# Autodesk Inventor assembly: Assembly1
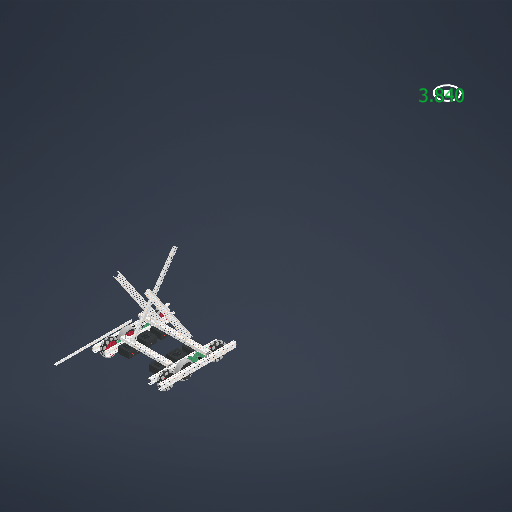
[picture p0: Inventor's stored thumbnail of the model, 512x512]
Saved by Autodesk Inventor 2026.2 (Build 302298000, 298)
## iProperties
Created: 2025-12-27
Part Number: Assembly1
Document SubType Name: Assembly
Designer: jacob
Author: jacob
## Documents named in this file (35)
- C:\Personal\Deprecated\VEX V5 Push Back\S-bot-two\CAD\Assembly1.iam
- C:\Personal\Deprecated\VEX V5 Push Back\S-bot-two\CAD\VEX-CAD-Inventor-1.4.2\Structure\C Channel\Aluminum 1x2x1\Alu C 1x2x1x30.ipt
- C:\Personal\Deprecated\VEX V5 Push Back\S-bot-two\CAD\VEX-CAD-Inventor-1.4.2\Structure\Hardware\Nut Nylock.ipt
- C:\Personal\Deprecated\VEX V5 Push Back\S-bot-two\CAD\VEX-CAD-Inventor-1.4.2\Motion\Spacers\Spacer Nylon .375 OD\NSpacer .375 OD x .500.ipt
- C:\Personal\Deprecated\VEX V5 Push Back\S-bot-two\CAD\VEX-CAD-Inventor-1.4.2\Motion\Spacers\Spacer Nylon .375 OD.ipt
- C:\Personal\Deprecated\VEX V5 Push Back\S-bot-two\CAD\VEX-CAD-Inventor-1.4.2\Motion\Wheels\Omni Wheel\3.25 Omni AS, No Insert.iam
- C:\Personal\Deprecated\VEX V5 Push Back\S-bot-two\CAD\VEX-CAD-Inventor-1.4.2\Motion\Wheels\Omni Wheel.iam
- C:\Personal\Deprecated\VEX V5 Push Back\S-bot-two\CAD\VEX-CAD-Inventor-1.4.2\Motion\HS Shaft Adapter Circle.ipt
- C:\Personal\Deprecated\VEX V5 Push Back\S-bot-two\CAD\VEX-CAD-Inventor-1.4.2\Motion\Wheels\Traction Wheel.iam
- C:\Personal\Deprecated\VEX V5 Push Back\S-bot-two\CAD\VEX-CAD-Inventor-1.4.2\Motion\Spacers\Spacer Nylon .375 OD\NSpacer .375 OD x .125.ipt
- C:\Personal\Deprecated\VEX V5 Push Back\S-bot-two\CAD\VEX-CAD-Inventor-1.4.2\Motion\Spacers\Washer Steel\SWasher .375 OD x .031250.ipt
- C:\Personal\Deprecated\VEX V5 Push Back\S-bot-two\CAD\VEX-CAD-Inventor-1.4.2\Motion\Spacers\Washer Steel.ipt
- C:\Personal\Deprecated\VEX V5 Push Back\S-bot-two\CAD\VEX-CAD-Inventor-1.4.2\Motion\Gears\HS Gear.iam
- C:\Personal\Deprecated\VEX V5 Push Back\S-bot-two\CAD\VEX-CAD-Inventor-1.4.2\Motion\Gears\HS Gear\HS 48T Gear, Circle.iam
- C:\Personal\Deprecated\VEX V5 Push Back\S-bot-two\CAD\VEX-CAD-Inventor-1.4.2\Motion\Gears\LS 36T Gear.ipt
- C:\Personal\Deprecated\VEX V5 Push Back\S-bot-two\CAD\VEX-CAD-Inventor-1.4.2\Structure\C Channel\Aluminum 1x2x1\Alu C 1x2x1x27.ipt
- C:\Personal\Deprecated\VEX V5 Push Back\S-bot-two\CAD\VEX-CAD-Inventor-1.4.2\Electronics\V5 Motor.ipt
- C:\Personal\Deprecated\VEX V5 Push Back\S-bot-two\CAD\VEX-CAD-Inventor-1.4.2\Motion\Shaft LS\Bearing Flat.ipt
- C:\Personal\Deprecated\VEX V5 Push Back\S-bot-two\CAD\VEX-CAD-Inventor-1.4.2\Motion\Spacers\Spacer Nylon .375 OD\NSpacer .375 OD x .250.ipt
- C:\Personal\Deprecated\VEX V5 Push Back\S-bot-two\CAD\VEX-CAD-Inventor-1.4.2\Motion\Wheels\Traction Wheel\3.25 Traction AS, Circle.iam
- C:\Personal\Deprecated\VEX V5 Push Back\S-bot-two\CAD\VEX-CAD-Inventor-1.4.2\Structure\Standoff.ipt
- C:\Personal\Deprecated\VEX V5 Push Back\S-bot-two\CAD\VEX-CAD-Inventor-1.4.2\Structure\Hardware\Nut Nylock_MIR.ipt
- C:\Personal\Deprecated\VEX V5 Push Back\S-bot-two\CAD\VEX-CAD-Inventor-1.4.2\Motion\HS Shaft Adapter Circle_MIR.ipt
- C:\Personal\Deprecated\VEX V5 Push Back\S-bot-two\CAD\VEX-CAD-Inventor-1.4.2\Motion\Gears\LS 36T Gear_MIR.ipt
- C:\Personal\Deprecated\VEX V5 Push Back\S-bot-two\CAD\VEX-CAD-Inventor-1.4.2\Electronics\V5 Motor_MIR.ipt
- C:\Personal\Deprecated\VEX V5 Push Back\S-bot-two\CAD\VEX-CAD-Inventor-1.4.2\Motion\Shaft LS\Bearing Flat_MIR.ipt
- C:\Personal\Deprecated\VEX V5 Push Back\S-bot-two\CAD\VEX-CAD-Inventor-1.4.2\Motion\Gears\HS Gear\HS 48T Gear, Circle_MIR.iam
- C:\Personal\Deprecated\VEX V5 Push Back\S-bot-two\CAD\VEX-CAD-Inventor-1.4.2\Motion\Wheels\Omni Wheel\3.25 Omni AS, No Insert_MIR.iam
- C:\Personal\Deprecated\VEX V5 Push Back\S-bot-two\CAD\VEX-CAD-Inventor-1.4.2\Motion\Wheels\Traction Wheel\3.25 Traction AS, Circle_MIR.iam
- C:\Personal\Deprecated\VEX V5 Push Back\S-bot-two\CAD\VEX-CAD-Inventor-1.4.2\Structure\Standoff\Standoff 1.00.ipt
- C:\Personal\Deprecated\VEX V5 Push Back\S-bot-two\CAD\VEX-CAD-Inventor-1.4.2\Structure\Standoff\Standoff .75.ipt
- C:\Personal\Deprecated\VEX V5 Push Back\S-bot-two\CAD\VEX-CAD-Inventor-1.4.2\Structure\C Channel\Aluminum 1x2x1\Alu C 1x2x1x19.ipt
- C:\Personal\Deprecated\VEX V5 Push Back\S-bot-two\CAD\VEX-CAD-Inventor-1.4.2\Structure\C Channel\Aluminum 1x2x1 Half\Alu Half C 1x2x1x2.ipt
- C:\Personal\Deprecated\VEX V5 Push Back\S-bot-two\CAD\VEX-CAD-Inventor-1.4.2\Structure\C Channel\Aluminum 1x2x1 Half\Alu Half C 1x2x1x30.ipt
- C:\Personal\Deprecated\VEX V5 Push Back\S-bot-two\CAD\VEX-CAD-Inventor-1.4.2\Game Objects\vex_Push_Back.ipt
## Components (115 placed, 28 different names)
1. Alu C 1x2x1x30:2 — Mate:1, Mate:2, Flush:1, Insert:44, Insert:45, Insert:62, Insert:130, Insert:131, Insert:132, Insert:133, Insert:134, Insert:135, Insert:266, Insert:457, Insert:459
2. Nut Nylock:2 — Insert:45, Insert:140
3. Nut Nylock:3 — Insert:44, Insert:137
4. Nut Nylock:4 — Insert:8, Insert:266
5. NSpacer .375 OD x .500:3 — Insert:8, Insert:101
6. HS Shaft Adapter Circle:5 — Insert:21, Insert:103, Insert:105
7. SWasher .375 OD x .031250:3 — Insert:21, Insert:102
8. SWasher .375 OD x .031250:5 — Insert:100, Insert:102
9. LS 36T Gear:1 — Insert:136
10. Alu C 1x2x1x27:1 — Insert:66, Insert:67, Insert:68, Insert:69, Insert:70, Insert:72, Insert:73, Insert:74, Insert:75, Insert:76, Insert:99, Insert:104, Insert:106, Insert:107, Insert:136, Insert:458, Insert:460, Insert:465, Insert:466, Insert:467, Insert:468, Insert:469, Insert:470, Insert:484, Insert:485
11. LS 36T Gear:7 — Insert:106
12. LS 36T Gear:8 — Insert:107
13. LS 36T Gear:9 — Insert:99, Rotation:1
14. Nut Nylock:5 — Insert:62, Insert:112
15. V5 Motor:1 — Insert:66, Insert:69, Insert:465, Insert:466
16. Bearing Flat:1 — Insert:67, Insert:72
17. V5 Motor:2 — Insert:68, Insert:70, Insert:469, Insert:470
18. Bearing Flat:2 — Insert:73, Insert:74
19. Bearing Flat:3 — Insert:75, Insert:76
20. SWasher .375 OD x .031250:13 — Insert:100, Insert:101
21. HS 48T Gear, Circle:3 [sub-assembly] — Insert:103, Rotation:1, Rotation:2
22. NSpacer .375 OD x .125:15 — Insert:104
23. 3.25 Omni AS, No Insert:4 [sub-assembly] — Insert:105, Rotation:2
24. NSpacer .375 OD x .500:16 — Insert:111, Insert:114
25. NSpacer .375 OD x .500:18 — Insert:111, Insert:112
26. NSpacer .375 OD x .250:20 — Insert:114, Insert:115
27. SWasher .375 OD x .031250:15 — Insert:115, Insert:116
28. SWasher .375 OD x .031250:16 — Insert:116, Insert:117
29. SWasher .375 OD x .031250:17 — Insert:117
30. NSpacer .375 OD x .500:21 — Insert:137
31. SWasher .375 OD x .031250:18 — Insert:122
32. SWasher .375 OD x .031250:19
33. SWasher .375 OD x .031250:20
34. HS 48T Gear, Circle:4 [sub-assembly] — Insert:121, Insert:123
35. NSpacer .375 OD x .125:22 — Insert:123
36. 3.25 Omni AS, No Insert:5 [sub-assembly] — Insert:121, Insert:122
37. NSpacer .375 OD x .500:23 — Insert:140
38. SWasher .375 OD x .031250:21 — Insert:139
39. SWasher .375 OD x .031250:22
40. SWasher .375 OD x .031250:23
41. HS 48T Gear, Circle:5 [sub-assembly] — Insert:138
42. NSpacer .375 OD x .125:24
43. Bearing Flat:4 — Insert:130, Insert:131
44. Bearing Flat:5 — Insert:132, Insert:133
45. Bearing Flat:6 — Insert:134, Insert:135
46. 3.25 Traction AS, Circle:1 [sub-assembly] — Insert:138, Insert:139
47. Alu C 1x2x1x30:3 — Insert:388, Insert:389, Insert:390, Insert:398, Insert:428, Insert:429, Insert:430, Insert:431, Insert:432, Insert:433, Insert:453, Insert:456, Insert:506, Insert:507
48. Nut Nylock_MIR:1 — Insert:388, Insert:423
49. Nut Nylock_MIR:2 — Insert:389, Insert:416
50. Nut Nylock_MIR:3 — Insert:390, Insert:391
51. NSpacer .375 OD x .500:34 — Insert:391, Insert:405
52. HS Shaft Adapter Circle_MIR:1 — Insert:392, Insert:407, Insert:409
53. SWasher .375 OD x .031250:36 — Insert:392, Insert:393
54. SWasher .375 OD x .031250:37 — Insert:393, Insert:406
55. Alu C 1x2x1x27:4 — Insert:395, Insert:396, Insert:397, Insert:399, Insert:400, Insert:401, Insert:402, Insert:403, Insert:404, Insert:408, Insert:447, Insert:448, Insert:449, Insert:450, Insert:451, Insert:452, Insert:454, Insert:482, Insert:483, Insert:508, Insert:509
56. LS 36T Gear_MIR:2 — Insert:395
57. LS 36T Gear_MIR:3 — Insert:396
58. LS 36T Gear_MIR:4 — Insert:397, Rotation:5
59. Nut Nylock_MIR:4 — Insert:398, Insert:410
60. V5 Motor_MIR:1 — Insert:447, Insert:448
61. Bearing Flat_MIR:1 — Insert:399, Insert:400
62. V5 Motor_MIR:2 — Insert:451, Insert:452
63. V5 Motor_MIR:3 — Insert:449, Insert:450
64. Bearing Flat_MIR:2 — Insert:401, Insert:402
65. Bearing Flat_MIR:3 — Insert:403, Insert:404
66. SWasher .375 OD x .031250:38 — Insert:405, Insert:406
67. HS 48T Gear, Circle_MIR:1 [sub-assembly] — Insert:407, Rotation:5, Rotation:6
68. NSpacer .375 OD x .125:35 — Insert:408
69. 3.25 Omni AS, No Insert_MIR:1 [sub-assembly] — Insert:409, Rotation:6
70. NSpacer .375 OD x .500:36 — Insert:411, Insert:412
71. NSpacer .375 OD x .500:37 — Insert:410, Insert:411
72. NSpacer .375 OD x .250:38 — Insert:412, Insert:413
73. SWasher .375 OD x .031250:39 — Insert:413, Insert:414
74. SWasher .375 OD x .031250:40 — Insert:414, Insert:415
75. SWasher .375 OD x .031250:41 — Insert:415
76. NSpacer .375 OD x .500:39 — Insert:416, Insert:418
77. SWasher .375 OD x .031250:42 — Insert:417, Insert:421
78. SWasher .375 OD x .031250:43 — Insert:417, Insert:419
79. SWasher .375 OD x .031250:44 — Insert:418, Insert:419
80. HS 48T Gear, Circle_MIR:2 [sub-assembly] — Insert:420, Insert:422
81. NSpacer .375 OD x .125:40 — Insert:420
82. 3.25 Omni AS, No Insert_MIR:2 [sub-assembly] — Insert:421, Insert:422
83. NSpacer .375 OD x .500:41 — Insert:423, Insert:425
84. SWasher .375 OD x .031250:45 — Insert:424, Insert:434
85. SWasher .375 OD x .031250:46 — Insert:424, Insert:426
86. SWasher .375 OD x .031250:47 — Insert:425, Insert:426
87. HS 48T Gear, Circle_MIR:3 [sub-assembly] — Insert:427, Insert:435
88. NSpacer .375 OD x .125:42 — Insert:427
89. Bearing Flat_MIR:4 — Insert:428, Insert:429
90. Bearing Flat_MIR:5 — Insert:430, Insert:431
91. Bearing Flat_MIR:6 — Insert:432, Insert:433
92. 3.25 Traction AS, Circle_MIR:1 [sub-assembly] — Insert:434, Insert:435
93. Standoff 1.00:20 — Insert:457, Insert:491
94. Standoff 1.00:21 — Insert:458, Insert:499
95. Standoff 1.00:22 — Insert:454, Insert:494
96. Standoff 1.00:23 — Insert:453, Insert:496, Insert:506
97. Standoff 1.00:24 — Insert:456, Insert:497, Insert:507
98. Standoff 1.00:25 — Insert:495, Insert:509
99. Standoff 1.00:26 — Insert:460, Insert:498
100. Standoff 1.00:27 — Insert:459, Insert:490
101. V5 Motor:3 — Insert:467, Insert:468
102. Standoff .75:28 — Insert:482, Insert:502, Insert:508
103. Standoff .75:29 — Insert:483, Insert:503
104. Standoff .75:30 — Insert:484, Insert:501
105. Standoff .75:31 — Insert:485, Insert:500
106. Alu C 1x2x1x27:3 — Insert:490, Insert:491, Insert:494, Insert:495, Insert:496, Insert:497, Insert:498, Insert:499, Insert:510, Insert:511, Insert:513, Insert:514
107. Alu C 1x2x1x19:1 — Insert:500, Insert:501, Insert:502, Insert:503, Insert:516, Insert:517
108. Alu C 1x2x1x30:4 — Insert:512
109. Alu Half C 1x2x1x2:4 — Insert:510, Insert:511, Insert:512
110. Alu Half C 1x2x1x2:5 — Insert:513, Insert:514, Insert:515
111. Alu C 1x2x1x30:5 — Insert:515
112. Alu Half C 1x2x1x2:6 — Insert:516, Insert:517, Insert:518
113. Alu Half C 1x2x1x30:1 — Insert:518
114. Alu Half C 1x2x1x30:2
115. vex_Push_Back:1
## Relationships (154: Insert 147, RelateRotation 4, Mate 2, Flush 1)
- Mate:1: Alu C 1x2x1x30:2
- Mate:2: Alu C 1x2x1x30:2
- Flush:1: Alu C 1x2x1x30:2
- Insert:8: Nut Nylock:4 ↔ NSpacer .375 OD x .500:3
- Insert:21: HS Shaft Adapter Circle:5 ↔ SWasher .375 OD x .031250:3
- Insert:44: Alu C 1x2x1x30:2 ↔ Nut Nylock:3
- Insert:45: Alu C 1x2x1x30:2 ↔ Nut Nylock:2
- Insert:62: Alu C 1x2x1x30:2 ↔ Nut Nylock:5
- Insert:66: Alu C 1x2x1x27:1 ↔ V5 Motor:1
- Insert:67: Alu C 1x2x1x27:1 ↔ Bearing Flat:1
- Insert:68: Alu C 1x2x1x27:1 ↔ V5 Motor:2
- Insert:69: Alu C 1x2x1x27:1 ↔ V5 Motor:1
- Insert:70: Alu C 1x2x1x27:1 ↔ V5 Motor:2
- Insert:72: Alu C 1x2x1x27:1 ↔ Bearing Flat:1
- Insert:73: Alu C 1x2x1x27:1 ↔ Bearing Flat:2
- Insert:74: Alu C 1x2x1x27:1 ↔ Bearing Flat:2
- Insert:75: Alu C 1x2x1x27:1 ↔ Bearing Flat:3
- Insert:76: Alu C 1x2x1x27:1 ↔ Bearing Flat:3
- Insert:99: Alu C 1x2x1x27:1 ↔ LS 36T Gear:9
- Insert:100: SWasher .375 OD x .031250:5 ↔ SWasher .375 OD x .031250:13
- Insert:101: NSpacer .375 OD x .500:3 ↔ SWasher .375 OD x .031250:13
- Insert:102: SWasher .375 OD x .031250:3 ↔ SWasher .375 OD x .031250:5
- Insert:103: HS Shaft Adapter Circle:5 ↔ HS 48T Gear, Circle:3
- Insert:104: Alu C 1x2x1x27:1 ↔ NSpacer .375 OD x .125:15
- Insert:105: HS Shaft Adapter Circle:5 ↔ 3.25 Omni AS, No Insert:4
- Insert:106: Alu C 1x2x1x27:1 ↔ LS 36T Gear:7
- Insert:107: Alu C 1x2x1x27:1 ↔ LS 36T Gear:8
- Insert:111: NSpacer .375 OD x .500:16 ↔ NSpacer .375 OD x .500:18
- Insert:112: Nut Nylock:5 ↔ NSpacer .375 OD x .500:18
- Insert:114: NSpacer .375 OD x .500:16 ↔ NSpacer .375 OD x .250:20
- Insert:115: NSpacer .375 OD x .250:20 ↔ SWasher .375 OD x .031250:15
- Insert:116: SWasher .375 OD x .031250:15 ↔ SWasher .375 OD x .031250:16
- Insert:117: SWasher .375 OD x .031250:16 ↔ SWasher .375 OD x .031250:17
- [Insert]: SWasher .375 OD x .031250:19 ↔ SWasher .375 OD x .031250:20
- [Insert]: NSpacer .375 OD x .500:21 ↔ SWasher .375 OD x .031250:20
- [Insert]: SWasher .375 OD x .031250:18 ↔ SWasher .375 OD x .031250:19
- Insert:121: HS 48T Gear, Circle:4 ↔ 3.25 Omni AS, No Insert:5
- Insert:122: SWasher .375 OD x .031250:18 ↔ 3.25 Omni AS, No Insert:5
- Insert:123: HS 48T Gear, Circle:4 ↔ NSpacer .375 OD x .125:22
- [Insert]: SWasher .375 OD x .031250:22 ↔ SWasher .375 OD x .031250:23
- [Insert]: NSpacer .375 OD x .500:23 ↔ SWasher .375 OD x .031250:23
- [Insert]: SWasher .375 OD x .031250:21 ↔ SWasher .375 OD x .031250:22
- [Insert]: HS 48T Gear, Circle:5 ↔ NSpacer .375 OD x .125:24
- Insert:130: Alu C 1x2x1x30:2 ↔ Bearing Flat:4
- Insert:131: Alu C 1x2x1x30:2 ↔ Bearing Flat:4
- Insert:132: Alu C 1x2x1x30:2 ↔ Bearing Flat:5
- Insert:133: Alu C 1x2x1x30:2 ↔ Bearing Flat:5
- Insert:134: Alu C 1x2x1x30:2 ↔ Bearing Flat:6
- Insert:135: Alu C 1x2x1x30:2 ↔ Bearing Flat:6
- Insert:136: LS 36T Gear:1 ↔ Alu C 1x2x1x27:1
- Insert:137: Nut Nylock:3 ↔ NSpacer .375 OD x .500:21
- Insert:138: HS 48T Gear, Circle:5 ↔ 3.25 Traction AS, Circle:1
- Insert:139: SWasher .375 OD x .031250:21 ↔ 3.25 Traction AS, Circle:1
- Insert:140: Nut Nylock:2 ↔ NSpacer .375 OD x .500:23
- Insert:266: Alu C 1x2x1x30:2 ↔ Nut Nylock:4
- Rotation:1 [RelateRotation] (1 ul): LS 36T Gear:9 ↔ HS 48T Gear, Circle:3
- Rotation:2 [RelateRotation] (1 ul): HS 48T Gear, Circle:3 ↔ 3.25 Omni AS, No Insert:4
- Insert:388: Alu C 1x2x1x30:3 ↔ Nut Nylock_MIR:1
- Insert:389: Alu C 1x2x1x30:3 ↔ Nut Nylock_MIR:2
- Insert:390: Alu C 1x2x1x30:3 ↔ Nut Nylock_MIR:3
- Insert:391: Nut Nylock_MIR:3 ↔ NSpacer .375 OD x .500:34
- Insert:392: HS Shaft Adapter Circle_MIR:1 ↔ SWasher .375 OD x .031250:36
- Insert:393: SWasher .375 OD x .031250:36 ↔ SWasher .375 OD x .031250:37
- Insert:395: Alu C 1x2x1x27:4 ↔ LS 36T Gear_MIR:2
- Insert:396: Alu C 1x2x1x27:4 ↔ LS 36T Gear_MIR:3
- Insert:397: Alu C 1x2x1x27:4 ↔ LS 36T Gear_MIR:4
- Insert:398: Alu C 1x2x1x30:3 ↔ Nut Nylock_MIR:4
- Insert:399: Alu C 1x2x1x27:4 ↔ Bearing Flat_MIR:1
- Insert:400: Alu C 1x2x1x27:4 ↔ Bearing Flat_MIR:1
- Insert:401: Alu C 1x2x1x27:4 ↔ Bearing Flat_MIR:2
- Insert:402: Alu C 1x2x1x27:4 ↔ Bearing Flat_MIR:2
- Insert:403: Alu C 1x2x1x27:4 ↔ Bearing Flat_MIR:3
- Insert:404: Alu C 1x2x1x27:4 ↔ Bearing Flat_MIR:3
- Insert:405: NSpacer .375 OD x .500:34 ↔ SWasher .375 OD x .031250:38
- Insert:406: SWasher .375 OD x .031250:37 ↔ SWasher .375 OD x .031250:38
- Insert:407: HS Shaft Adapter Circle_MIR:1 ↔ HS 48T Gear, Circle_MIR:1
- Rotation:5 [RelateRotation] (1 ul): LS 36T Gear_MIR:4 ↔ HS 48T Gear, Circle_MIR:1
- Insert:408: Alu C 1x2x1x27:4 ↔ NSpacer .375 OD x .125:35
- Insert:409: HS Shaft Adapter Circle_MIR:1 ↔ 3.25 Omni AS, No Insert_MIR:1
- Rotation:6 [RelateRotation] (1 ul): HS 48T Gear, Circle_MIR:1 ↔ 3.25 Omni AS, No Insert_MIR:1
- Insert:410: Nut Nylock_MIR:4 ↔ NSpacer .375 OD x .500:37
- Insert:411: NSpacer .375 OD x .500:36 ↔ NSpacer .375 OD x .500:37
- Insert:412: NSpacer .375 OD x .500:36 ↔ NSpacer .375 OD x .250:38
- Insert:413: NSpacer .375 OD x .250:38 ↔ SWasher .375 OD x .031250:39
- Insert:414: SWasher .375 OD x .031250:39 ↔ SWasher .375 OD x .031250:40
- Insert:415: SWasher .375 OD x .031250:40 ↔ SWasher .375 OD x .031250:41
- Insert:416: Nut Nylock_MIR:2 ↔ NSpacer .375 OD x .500:39
- Insert:417: SWasher .375 OD x .031250:42 ↔ SWasher .375 OD x .031250:43
- Insert:418: NSpacer .375 OD x .500:39 ↔ SWasher .375 OD x .031250:44
- Insert:419: SWasher .375 OD x .031250:43 ↔ SWasher .375 OD x .031250:44
- Insert:420: HS 48T Gear, Circle_MIR:2 ↔ NSpacer .375 OD x .125:40
- Insert:421: SWasher .375 OD x .031250:42 ↔ 3.25 Omni AS, No Insert_MIR:2
- Insert:422: HS 48T Gear, Circle_MIR:2 ↔ 3.25 Omni AS, No Insert_MIR:2
- Insert:423: Nut Nylock_MIR:1 ↔ NSpacer .375 OD x .500:41
- Insert:424: SWasher .375 OD x .031250:45 ↔ SWasher .375 OD x .031250:46
- Insert:425: NSpacer .375 OD x .500:41 ↔ SWasher .375 OD x .031250:47
- Insert:426: SWasher .375 OD x .031250:46 ↔ SWasher .375 OD x .031250:47
- Insert:427: HS 48T Gear, Circle_MIR:3 ↔ NSpacer .375 OD x .125:42
- Insert:428: Alu C 1x2x1x30:3 ↔ Bearing Flat_MIR:4
- Insert:429: Alu C 1x2x1x30:3 ↔ Bearing Flat_MIR:4
- Insert:430: Alu C 1x2x1x30:3 ↔ Bearing Flat_MIR:5
- Insert:431: Alu C 1x2x1x30:3 ↔ Bearing Flat_MIR:5
- Insert:432: Alu C 1x2x1x30:3 ↔ Bearing Flat_MIR:6
- Insert:433: Alu C 1x2x1x30:3 ↔ Bearing Flat_MIR:6
- Insert:434: SWasher .375 OD x .031250:45 ↔ 3.25 Traction AS, Circle_MIR:1
- Insert:435: HS 48T Gear, Circle_MIR:3 ↔ 3.25 Traction AS, Circle_MIR:1
- Insert:447: Alu C 1x2x1x27:4 ↔ V5 Motor_MIR:1
- Insert:448: Alu C 1x2x1x27:4 ↔ V5 Motor_MIR:1
- Insert:449: Alu C 1x2x1x27:4 ↔ V5 Motor_MIR:3
- Insert:450: Alu C 1x2x1x27:4 ↔ V5 Motor_MIR:3
- Insert:451: Alu C 1x2x1x27:4 ↔ V5 Motor_MIR:2
- Insert:452: Alu C 1x2x1x27:4 ↔ V5 Motor_MIR:2
- Insert:453: Alu C 1x2x1x30:3 ↔ Standoff 1.00:23
- Insert:454: Alu C 1x2x1x27:4 ↔ Standoff 1.00:22
- Insert:456: Alu C 1x2x1x30:3 ↔ Standoff 1.00:24
- Insert:457: Alu C 1x2x1x30:2 ↔ Standoff 1.00:20
- Insert:458: Alu C 1x2x1x27:1 ↔ Standoff 1.00:21
- Insert:459: Alu C 1x2x1x30:2 ↔ Standoff 1.00:27
- Insert:460: Alu C 1x2x1x27:1 ↔ Standoff 1.00:26
- Insert:465: Alu C 1x2x1x27:1 ↔ V5 Motor:1
- Insert:466: Alu C 1x2x1x27:1 ↔ V5 Motor:1
- Insert:467: Alu C 1x2x1x27:1 ↔ V5 Motor:3
- Insert:468: Alu C 1x2x1x27:1 ↔ V5 Motor:3
- Insert:469: Alu C 1x2x1x27:1 ↔ V5 Motor:2
- Insert:470: Alu C 1x2x1x27:1 ↔ V5 Motor:2
- Insert:482: Alu C 1x2x1x27:4 ↔ Standoff .75:28
- Insert:483: Alu C 1x2x1x27:4 ↔ Standoff .75:29
- Insert:484: Alu C 1x2x1x27:1 ↔ Standoff .75:30
- Insert:485: Alu C 1x2x1x27:1 ↔ Standoff .75:31
- Insert:490: Standoff 1.00:27 ↔ Alu C 1x2x1x27:3
- Insert:491: Standoff 1.00:20 ↔ Alu C 1x2x1x27:3
- Insert:494: Standoff 1.00:22 ↔ Alu C 1x2x1x27:3
- Insert:495: Standoff 1.00:25 ↔ Alu C 1x2x1x27:3
- Insert:496: Standoff 1.00:23 ↔ Alu C 1x2x1x27:3
- Insert:497: Standoff 1.00:24 ↔ Alu C 1x2x1x27:3
- Insert:498: Standoff 1.00:26 ↔ Alu C 1x2x1x27:3
- Insert:499: Standoff 1.00:21 ↔ Alu C 1x2x1x27:3
- Insert:500: Standoff .75:31 ↔ Alu C 1x2x1x19:1
- Insert:501: Standoff .75:30 ↔ Alu C 1x2x1x19:1
- Insert:502: Standoff .75:28 ↔ Alu C 1x2x1x19:1
- Insert:503: Standoff .75:29 ↔ Alu C 1x2x1x19:1
- Insert:506: Alu C 1x2x1x30:3 ↔ Standoff 1.00:23
- Insert:507: Alu C 1x2x1x30:3 ↔ Standoff 1.00:24
- Insert:508: Alu C 1x2x1x27:4 ↔ Standoff .75:28
- Insert:509: Alu C 1x2x1x27:4 ↔ Standoff 1.00:25
- Insert:510: Alu C 1x2x1x27:3 ↔ Alu Half C 1x2x1x2:4
- Insert:511: Alu C 1x2x1x27:3 ↔ Alu Half C 1x2x1x2:4
- Insert:512: Alu C 1x2x1x30:4 ↔ Alu Half C 1x2x1x2:4
- Insert:513: Alu C 1x2x1x27:3 ↔ Alu Half C 1x2x1x2:5
- Insert:514: Alu C 1x2x1x27:3 ↔ Alu Half C 1x2x1x2:5
- Insert:515: Alu Half C 1x2x1x2:5 ↔ Alu C 1x2x1x30:5
- Insert:516: Alu C 1x2x1x19:1 ↔ Alu Half C 1x2x1x2:6
- Insert:517: Alu C 1x2x1x19:1 ↔ Alu Half C 1x2x1x2:6
- Insert:518: Alu Half C 1x2x1x2:6 ↔ Alu Half C 1x2x1x30:1
## Named parameters: d162_d144 = 0 mm, d163_d145 = 0 mm, d164_d146 = 0 mm, d168_d162_d144 = 0 mm, d169_d163_d145 = 0 mm, d170_d164_d146 = 0 mm, d173_d167 = 0 mm
